# Autodesk Inventor assembly: TankFlipper
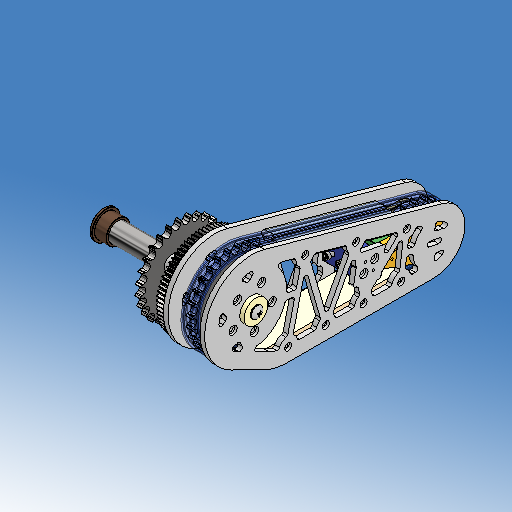
[picture p0: Inventor's stored thumbnail of the model, 512x512]
Saved by Autodesk Inventor 2025 (Build 290162000, 162)
## iProperties
Created: 2024-02-14
Part Number: TankFlipper
Document SubType Name: Assembly
Designer: seene
Author: seene
## Documents named in this file (8)
- C:\Users\seene\Desktop\Stony Brook\SBRT\RCR_Dexter\Drive\v1\TankFlipper.iam
- C:\Users\seene\Desktop\Stony Brook\SBRT\RCR_Dexter\Drive\v1\TANK flipper\panel_outside.ipt
- C:\Users\seene\Desktop\Stony Brook\SBRT\RCR_Dexter\Drive\v1\TANK flipper\panel_inside.ipt
- C:\Users\seene\Desktop\Stony Brook\SBRT\RCR_Dexter\Drive\v1\TANK flipper\flat chain guide.ipt
- C:\Users\seene\Desktop\Stony Brook\SBRT\RCR_Dexter\Drive\v1\TANK flipper\chain guide.ipt
- C:\Users\seene\Desktop\Stony Brook\SBRT\RCR_Dexter\Drive\v1\TANK flipper\TankFlipperAssembledDriveShaft.iam
- C:\Users\seene\Desktop\Stony Brook\SBRT\RCR_Dexter\Drive\v1\TANK flipper\flipper_tensioner _belt.iam
- C:\Users\seene\Desktop\Stony Brook\SBRT\RCR_Dexter\Drive\v1\TankFlipper\Design Accelerator\Chain Drive1.iam
## Components (7 placed, 7 different names)
1. panel_outside:1 — Mate:1, Mate:2, Mate:3, Rigid:2
2. panel_inside:1 — Mate:4, Mate:5, Mate:6, Mate:9, Mate:10, Mate:15, Mate:16, Mate:17
3. flat chain guide:1 — Mate:1, Mate:2, Mate:3, Mate:4, Mate:5, Mate:10
4. chain guide:1 — Mate:6, Mate:9
5. TankFlipperAssembledDriveShaft:1 [sub-assembly] — Rigid:2
6. flipper_tensioner _belt:1 [sub-assembly] — Mate:15, Mate:16, Mate:17
7. Chain Drive:1 [sub-assembly]
## Relationships (12: Mate 11, WeldJoint 1)
- Mate:1: panel_outside:1 ↔ flat chain guide:1
- Mate:2: panel_outside:1 ↔ flat chain guide:1
- Mate:3: panel_outside:1 ↔ flat chain guide:1
- Mate:4: panel_inside:1 ↔ flat chain guide:1
- Mate:5: panel_inside:1 ↔ flat chain guide:1
- Mate:6: panel_inside:1 ↔ chain guide:1
- Mate:9: panel_inside:1 ↔ chain guide:1
- Mate:10: panel_inside:1 ↔ flat chain guide:1
- Rigid:2 [WeldJoint]: panel_outside:1 ↔ TankFlipperAssembledDriveShaft:1
- Mate:15: panel_inside:1 ↔ flipper_tensioner _belt:1
- Mate:16: panel_inside:1 ↔ flipper_tensioner _belt:1
- Mate:17: panel_inside:1 ↔ flipper_tensioner _belt:1
